# Autodesk Inventor assembly: Outer
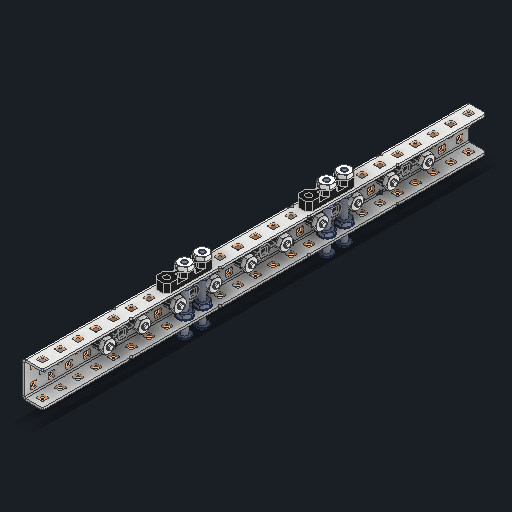
[picture p0: Inventor's stored thumbnail of the model, 512x512]
Saved by Autodesk Inventor 2025.1 (Build 291241000, 241)
## iProperties
Created: 2024-11-28
Part Number: Outer
Document SubType Name: Assembly
Designer: avere
Author: avere
## Documents named in this file (10)
- C:\Users\avere\VEX\High Stakes\CAD\Codie\Chassis\Drivebay Left\Outer.iam
- C:\Users\avere\VEX\High Stakes\CAD\ROBOPROS-CAD-Inventor\Structure\C Channel\Aluminum 1x2x1\Alu C 1x2x1x25.ipt
- C:\Users\avere\VEX\High Stakes\CAD\Codie\Chassis\Drivebay Left\Gear Layout.ipt
- C:\Users\avere\VEX\High Stakes\CAD\ROBOPROS-CAD-Inventor\Quick Assemblies\Bearing Flat NScrew Slotted.iam
- C:\Users\avere\VEX\High Stakes\CAD\ROBOPROS-CAD-Inventor\Structure\Hardware\Nut Keps.ipt
- C:\Users\avere\VEX\High Stakes\CAD\ROBOPROS-CAD-Inventor\Motion\Shaft LS\Bearing Flat.ipt
- C:\Users\avere\VEX\High Stakes\CAD\ROBOPROS-CAD-Inventor\Structure\Hardware\Nut Nylon\Nut Nylon - White.ipt
- C:\Users\avere\VEX\High Stakes\CAD\ROBOPROS-CAD-Inventor\Structure\Hardware\Nut Nylon.ipt
- C:\Users\avere\VEX\High Stakes\CAD\ROBOPROS-CAD-Inventor\Structure\Hardware\Screw Steel - Star\SScrew Star Smooth 1.750.ipt
- C:\Users\avere\VEX\High Stakes\CAD\ROBOPROS-CAD-Inventor\Structure\Hardware\Screw Steel - Star.ipt
## Components (25 placed, 7 different names)
1. Alu C 1x2x1x25:1 — Flush:1, Flush:2, Mate:1, Mate:4, Mate:5, Insert:1, Mate:6, Insert:4, Insert:5, Insert:6, Insert:7, Insert:8, Mate:7, Insert:11, Insert:12
2. Gear Layout:1 — Mate:4, Mate:5
3. Bearing Flat NScrew Slotted:1 [sub-assembly] — Insert:1, Mate:6
4. Bearing Flat NScrew Slotted:2 [sub-assembly]
5. Bearing Flat NScrew Slotted:3 [sub-assembly]
6. Bearing Flat NScrew Slotted:4 [sub-assembly]
7. Bearing Flat NScrew Slotted:5 [sub-assembly]
8. Nut Keps:1 — Insert:7
9. Nut Keps:2 — Insert:6
10. Nut Keps:3 — Insert:5
11. Nut Keps:4 — Insert:4
12. Bearing Flat:1 — Insert:8, Mate:7, Insert:9, Insert:10
13. Nut Nylon - White:1 — Insert:10
14. Nut Nylon - White:2 — Insert:9
15. SScrew Star Smooth 1.750:1 — Insert:12
16. SScrew Star Smooth 1.750:2 — Insert:11
17. Nut Keps:5
18. Nut Keps:6
19. Nut Keps:7
20. Nut Keps:8
21. Bearing Flat:2
22. Nut Nylon - White:3
23. Nut Nylon - White:4
24. SScrew Star Smooth 1.750:3
25. SScrew Star Smooth 1.750:4
## Component patterns: Bearings (5 elements), (2 elements, first: Nut Keps:1 + Nut Keps:2 + Nut Keps:3 + Nut Keps:4 + Bearing Flat:1 + Nut Nylon - White:1 + Nut Nylon - White:2 + SScrew Star Smooth 1.750:1 + SScrew Star Smooth 1.750:2)
## Relationships (17: Insert 10, Mate 5, Flush 2)
- Flush:1 (-158.75 mm): Alu C 1x2x1x25:1
- Flush:2 (-12.7 mm): Alu C 1x2x1x25:1
- Mate:1: Alu C 1x2x1x25:1
- Mate:4: Alu C 1x2x1x25:1 ↔ Gear Layout:1
- Mate:5: Alu C 1x2x1x25:1 ↔ Gear Layout:1
- Insert:1: Alu C 1x2x1x25:1 ↔ Bearing Flat NScrew Slotted:1
- Mate:6: Alu C 1x2x1x25:1 ↔ Bearing Flat NScrew Slotted:1
- Insert:4: Alu C 1x2x1x25:1 ↔ Nut Keps:4
- Insert:5: Alu C 1x2x1x25:1 ↔ Nut Keps:3
- Insert:6: Alu C 1x2x1x25:1 ↔ Nut Keps:2
- Insert:7: Alu C 1x2x1x25:1 ↔ Nut Keps:1
- Insert:8: Alu C 1x2x1x25:1 ↔ Bearing Flat:1
- Mate:7: Alu C 1x2x1x25:1 ↔ Bearing Flat:1
- Insert:9: Bearing Flat:1 ↔ Nut Nylon - White:2
- Insert:10: Bearing Flat:1 ↔ Nut Nylon - White:1
- Insert:11 (9.525 mm): Alu C 1x2x1x25:1 ↔ SScrew Star Smooth 1.750:2
- Insert:12 (9.525 mm): Alu C 1x2x1x25:1 ↔ SScrew Star Smooth 1.750:1
